# Autodesk Inventor assembly: КВ33.000.100 - Блок переключение передач
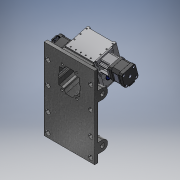
[picture p0: Inventor's stored thumbnail of the model, 180x180]
Saved by Autodesk Inventor 2019 (Build 230136000, 136)
## iProperties
Created: 2021-02-22
Part Number: КВ33.000.100 - Блок переключение передач
Material: Типовые
Document SubType Name: Assembly
Designer: Петров Иван
Author: Петров Иван
## Documents named in this file (14)
- E:\IVAN\Ivan_desktop\Kvantorium\Projects\tractor\design\КВ33.000.100 - Блок переключение передач.iam
- E:\IVAN\Ivan_desktop\Kvantorium\Projects\tractor\design\design_models\крышка КП.ipt
- E:\IVAN\Ivan_desktop\Kvantorium\Projects\tractor\design\КВ33.000.101 - Площадка крепежная.ipt
- E:\IVAN\Ivan_desktop\Kvantorium\Projects\tractor\design\КВ33.000.102 - Стенка толстая.ipt
- E:\IVAN\Ivan_desktop\Kvantorium\Projects\tractor\design\КВ33.000.103 - Стенка тонкая.ipt
- C:\Users\Петров Иван\Documents\Inventor\Content Center Files\R2019\en-US\GOST 9649-78\Washer 3 GOST 9649-78.ipt
- C:\Users\Петров Иван\Documents\Inventor\Content Center Files\R2019\en-US\Screw A2 GOST 17473-80\Screw A2.M2.5-6gx7 GOST 17473-80.ipt
- E:\IVAN\Ivan_desktop\Kvantorium\Projects\tractor\design\КВ33.000.104 - Крышка.ipt
- E:\IVAN\Ivan_desktop\Kvantorium\Projects\tractor\design\standart_components\Вал.ipt
- E:\IVAN\Ivan_desktop\Kvantorium\Projects\tractor\design\standart_components\Подшипник 626Z.ipt
- E:\IVAN\Ivan_desktop\Kvantorium\Projects\tractor\design\КВ33.000.105 - Заслонка.ipt
- E:\IVAN\Ivan_desktop\Kvantorium\Projects\tractor\design\standart_components\nema 17 motor.ipt
- E:\IVAN\Ivan_desktop\Kvantorium\Projects\tractor\design\КВ33.000.106 - Муфта.ipt
- E:\IVAN\Ivan_desktop\Kvantorium\Projects\tractor\design\КВ33.000.107 - Крепеж мотора.ipt
## Components (74 placed, 13 different names)
1. крышка КП:1 — Mate:1, Mate:8, Mate:9
2. КВ33.000.101 - Площадка крепежная:1 — Mate:1, Mate:3, Angle:1, Mate:4, Mate:6, Mate:8, Mate:9, Mate:21, Mate:27, Mate:28, Mate:37
3. КВ33.000.102 - Стенка толстая:1 — Mate:3, Angle:1, Insert:6, Insert:7, Insert:8, Insert:9, Insert:10, Mate:14, Mate:15, Mate:16, Mate:17, Mate:20, Mate:23, Mate:25, Mate:26, Mate:38, Angle:2, Mate:47
4. КВ33.000.102 - Стенка толстая:2 — Mate:4, Insert:1, Insert:2, Insert:3, Insert:4, Insert:5, Flush:4, Mate:10, Mate:11, Mate:12, Mate:13, Flush:5, Mate:28, Mate:37, Mate:42
5. КВ33.000.103 - Стенка тонкая:2 — Mate:6, Insert:22, Insert:23, Insert:24, Insert:25, Insert:26, Insert:27, Insert:28, Insert:29, Insert:30, Insert:31, Insert:32, Mate:21, Mate:38, Flush:10
6. КВ33.000.104 - Крышка:1 — Flush:4
7. Подшипник 626Z:1 — Mate:10, Mate:11, Mate:18
8. Подшипник 626Z:2 — Mate:14, Mate:15
9. Подшипник 626Z:3 — Mate:16, Mate:17
10. Подшипник 626Z:4 — Mate:12, Mate:13, Mate:19
11. Вал:1 — Mate:18, Flush:5, Flush:6, Mate:31, Mate:40, Rotation:2
12. Вал:2 — Mate:19, Flush:6, Mate:22, Mate:29, Mate:30, Rotation:1
13. КВ33.000.105 - Заслонка:1 — Mate:20
14. nema 17 motor:1 — Mate:22, Mate:23, Mate:48
15. nema 17 motor:2 — Mate:43, Mate:44, Mate:45
16. КВ33.000.103 - Стенка тонкая:3 — Mate:25, Mate:26, Mate:27, Flush:11
17. КВ33.000.106 - Муфта:1 — Mate:29, Mate:30, Mate:46, Rotation:1
18. КВ33.000.106 - Муфта:2 — Mate:31, Mate:40, Mate:41, Rotation:2
19. КВ33.000.107 - Крепеж мотора:1 — Angle:2, Flush:11, Mate:46, Mate:47, Mate:48
20. КВ33.000.107 - Крепеж мотора:2 — Mate:41, Mate:42, Flush:10, Mate:43, Mate:44, Mate:45
21. Washer GOST 9649-78 3:1 — Insert:1, Insert:49
22. Washer GOST 9649-78 3:2 — Insert:2, Insert:50
23. Washer GOST 9649-78 3:3 — Insert:3, Insert:51
24. Washer GOST 9649-78 3:4 — Insert:4, Insert:52
25. Washer GOST 9649-78 3:5 — Insert:5, Insert:53
26. Washer GOST 9649-78 3:6 — Insert:6, Insert:33
27. Washer GOST 9649-78 3:7 — Insert:7, Insert:34
28. Washer GOST 9649-78 3:8 — Insert:8, Insert:35
29. Washer GOST 9649-78 3:9 — Insert:9, Insert:36
30. Washer GOST 9649-78 3:10 — Insert:10, Insert:37
31. Washer GOST 9649-78 3:11 — Insert:42
32. Washer GOST 9649-78 3:12 — Insert:40
33. Washer GOST 9649-78 3:13 — Insert:41
34. Washer GOST 9649-78 3:14 — Insert:39
35. Washer GOST 9649-78 3:15 — Insert:38
36. Washer GOST 9649-78 3:16 — Insert:45
37. Washer GOST 9649-78 3:17 — Insert:44
38. Washer GOST 9649-78 3:18 — Insert:43
39. Washer GOST 9649-78 3:19 — Insert:46
40. Washer GOST 9649-78 3:20 — Insert:47
41. Washer GOST 9649-78 3:21 — Insert:48
42. Washer GOST 9649-78 3:22 — Insert:22
43. Washer GOST 9649-78 3:23 — Insert:23
44. Washer GOST 9649-78 3:24 — Insert:24
45. Washer GOST 9649-78 3:25 — Insert:25
46. Washer GOST 9649-78 3:26 — Insert:26
47. Washer GOST 9649-78 3:27 — Insert:27
48. Washer GOST 9649-78 3:28 — Insert:28
49. Washer GOST 9649-78 3:29 — Insert:29
50. Washer GOST 9649-78 3:30 — Insert:30, Insert:54
51. Washer GOST 9649-78 3:31 — Insert:31
52. Washer GOST 9649-78 3:32 — Insert:32
53. Screw A2 GOST 17473-80 M2.5-6gx7:1 — Insert:33
54. Screw A2 GOST 17473-80 M2.5-6gx7:2 — Insert:34
55. Screw A2 GOST 17473-80 M2.5-6gx7:3 — Insert:35
56. Screw A2 GOST 17473-80 M2.5-6gx7:4 — Insert:36
57. Screw A2 GOST 17473-80 M2.5-6gx7:5 — Insert:37
58. Screw A2 GOST 17473-80 M2.5-6gx7:6 — Insert:38
59. Screw A2 GOST 17473-80 M2.5-6gx7:7 — Insert:39
60. Screw A2 GOST 17473-80 M2.5-6gx7:8 — Insert:40
61. Screw A2 GOST 17473-80 M2.5-6gx7:9 — Insert:41
62. Screw A2 GOST 17473-80 M2.5-6gx7:10 — Insert:42
63. Screw A2 GOST 17473-80 M2.5-6gx7:11 — Insert:43
64. Screw A2 GOST 17473-80 M2.5-6gx7:12 — Insert:44
65. Screw A2 GOST 17473-80 M2.5-6gx7:13 — Insert:45
66. Screw A2 GOST 17473-80 M2.5-6gx7:14 — Insert:46
67. Screw A2 GOST 17473-80 M2.5-6gx7:15 — Insert:47
68. Screw A2 GOST 17473-80 M2.5-6gx7:16 — Insert:48
69. Screw A2 GOST 17473-80 M2.5-6gx7:17 — Insert:49
70. Screw A2 GOST 17473-80 M2.5-6gx7:18 — Insert:50
71. Screw A2 GOST 17473-80 M2.5-6gx7:19 — Insert:51
72. Screw A2 GOST 17473-80 M2.5-6gx7:20 — Insert:52
73. Screw A2 GOST 17473-80 M2.5-6gx7:21 — Insert:53
74. Screw A2 GOST 17473-80 M2.5-6gx7:22 — Insert:54
## Relationships (90: Insert 43, Mate 38, Flush 5, Angle 2, RelateRotation 2)
- Mate:1: крышка КП:1 ↔ КВ33.000.101 - Площадка крепежная:1
- Mate:3: КВ33.000.101 - Площадка крепежная:1 ↔ КВ33.000.102 - Стенка толстая:1
- Angle:1 (0 deg): КВ33.000.101 - Площадка крепежная:1 ↔ КВ33.000.102 - Стенка толстая:1
- Mate:4: КВ33.000.101 - Площадка крепежная:1 ↔ КВ33.000.102 - Стенка толстая:2
- Mate:6: КВ33.000.101 - Площадка крепежная:1 ↔ КВ33.000.103 - Стенка тонкая:2
- Insert:1: КВ33.000.102 - Стенка толстая:2 ↔ Washer GOST 9649-78 3:1
- Insert:2: КВ33.000.102 - Стенка толстая:2 ↔ Washer GOST 9649-78 3:2
- Insert:3: КВ33.000.102 - Стенка толстая:2 ↔ Washer GOST 9649-78 3:3
- Insert:4: КВ33.000.102 - Стенка толстая:2 ↔ Washer GOST 9649-78 3:4
- Insert:5: КВ33.000.102 - Стенка толстая:2 ↔ Washer GOST 9649-78 3:5
- Insert:6: КВ33.000.102 - Стенка толстая:1 ↔ Washer GOST 9649-78 3:6
- Insert:7: КВ33.000.102 - Стенка толстая:1 ↔ Washer GOST 9649-78 3:7
- Insert:8: КВ33.000.102 - Стенка толстая:1 ↔ Washer GOST 9649-78 3:8
- Insert:9: КВ33.000.102 - Стенка толстая:1 ↔ Washer GOST 9649-78 3:9
- Insert:10: КВ33.000.102 - Стенка толстая:1 ↔ Washer GOST 9649-78 3:10
- Insert:22: КВ33.000.103 - Стенка тонкая:2 ↔ Washer GOST 9649-78 3:22
- Insert:23: КВ33.000.103 - Стенка тонкая:2 ↔ Washer GOST 9649-78 3:23
- Insert:24: КВ33.000.103 - Стенка тонкая:2 ↔ Washer GOST 9649-78 3:24
- Insert:25: КВ33.000.103 - Стенка тонкая:2 ↔ Washer GOST 9649-78 3:25
- Insert:26: КВ33.000.103 - Стенка тонкая:2 ↔ Washer GOST 9649-78 3:26
- Insert:27: КВ33.000.103 - Стенка тонкая:2 ↔ Washer GOST 9649-78 3:27
- Insert:28: КВ33.000.103 - Стенка тонкая:2 ↔ Washer GOST 9649-78 3:28
- Insert:29: КВ33.000.103 - Стенка тонкая:2 ↔ Washer GOST 9649-78 3:29
- Insert:30: КВ33.000.103 - Стенка тонкая:2 ↔ Washer GOST 9649-78 3:30
- Insert:31: КВ33.000.103 - Стенка тонкая:2 ↔ Washer GOST 9649-78 3:31
- Insert:32: КВ33.000.103 - Стенка тонкая:2 ↔ Washer GOST 9649-78 3:32
- Insert:33: Washer GOST 9649-78 3:6 ↔ Screw A2 GOST 17473-80 M2.5-6gx7:1
- Insert:34: Washer GOST 9649-78 3:7 ↔ Screw A2 GOST 17473-80 M2.5-6gx7:2
- Insert:35: Washer GOST 9649-78 3:8 ↔ Screw A2 GOST 17473-80 M2.5-6gx7:3
- Insert:36: Washer GOST 9649-78 3:9 ↔ Screw A2 GOST 17473-80 M2.5-6gx7:4
- Insert:37: Washer GOST 9649-78 3:10 ↔ Screw A2 GOST 17473-80 M2.5-6gx7:5
- Insert:38: Washer GOST 9649-78 3:15 ↔ Screw A2 GOST 17473-80 M2.5-6gx7:6
- Insert:39: Washer GOST 9649-78 3:14 ↔ Screw A2 GOST 17473-80 M2.5-6gx7:7
- Insert:40: Washer GOST 9649-78 3:12 ↔ Screw A2 GOST 17473-80 M2.5-6gx7:8
- Insert:41: Washer GOST 9649-78 3:13 ↔ Screw A2 GOST 17473-80 M2.5-6gx7:9
- Insert:42: Washer GOST 9649-78 3:11 ↔ Screw A2 GOST 17473-80 M2.5-6gx7:10
- Insert:43: Washer GOST 9649-78 3:18 ↔ Screw A2 GOST 17473-80 M2.5-6gx7:11
- Insert:44: Washer GOST 9649-78 3:17 ↔ Screw A2 GOST 17473-80 M2.5-6gx7:12
- Insert:45: Washer GOST 9649-78 3:16 ↔ Screw A2 GOST 17473-80 M2.5-6gx7:13
- Insert:46: Washer GOST 9649-78 3:19 ↔ Screw A2 GOST 17473-80 M2.5-6gx7:14
- Insert:47: Washer GOST 9649-78 3:20 ↔ Screw A2 GOST 17473-80 M2.5-6gx7:15
- Insert:48: Washer GOST 9649-78 3:21 ↔ Screw A2 GOST 17473-80 M2.5-6gx7:16
- Insert:49: Washer GOST 9649-78 3:1 ↔ Screw A2 GOST 17473-80 M2.5-6gx7:17
- Insert:50: Washer GOST 9649-78 3:2 ↔ Screw A2 GOST 17473-80 M2.5-6gx7:18
- Insert:51: Washer GOST 9649-78 3:3 ↔ Screw A2 GOST 17473-80 M2.5-6gx7:19
- Insert:52: Washer GOST 9649-78 3:4 ↔ Screw A2 GOST 17473-80 M2.5-6gx7:20
- Insert:53: Washer GOST 9649-78 3:5 ↔ Screw A2 GOST 17473-80 M2.5-6gx7:21
- Insert:54: Washer GOST 9649-78 3:30 ↔ Screw A2 GOST 17473-80 M2.5-6gx7:22
- Flush:4: КВ33.000.102 - Стенка толстая:2 ↔ КВ33.000.104 - Крышка:1
- Mate:8: крышка КП:1 ↔ КВ33.000.101 - Площадка крепежная:1
- Mate:9: крышка КП:1 ↔ КВ33.000.101 - Площадка крепежная:1
- Mate:10: КВ33.000.102 - Стенка толстая:2 ↔ Подшипник 626Z:1
- Mate:11: КВ33.000.102 - Стенка толстая:2 ↔ Подшипник 626Z:1
- Mate:12: КВ33.000.102 - Стенка толстая:2 ↔ Подшипник 626Z:4
- Mate:13: КВ33.000.102 - Стенка толстая:2 ↔ Подшипник 626Z:4
- Mate:14: КВ33.000.102 - Стенка толстая:1 ↔ Подшипник 626Z:2
- Mate:15: КВ33.000.102 - Стенка толстая:1 ↔ Подшипник 626Z:2
- Mate:16: КВ33.000.102 - Стенка толстая:1 ↔ Подшипник 626Z:3
- Mate:17: КВ33.000.102 - Стенка толстая:1 ↔ Подшипник 626Z:3
- Mate:18: Подшипник 626Z:1 ↔ Вал:1
- Flush:5 (-7.5 mm): КВ33.000.102 - Стенка толстая:2 ↔ Вал:1
- Mate:19: Подшипник 626Z:4 ↔ Вал:2
- Flush:6: Вал:1 ↔ Вал:2
- Mate:20: КВ33.000.102 - Стенка толстая:1 ↔ КВ33.000.105 - Заслонка:1
- Mate:21: КВ33.000.101 - Площадка крепежная:1 ↔ КВ33.000.103 - Стенка тонкая:2
- Mate:22: Вал:2 ↔ nema 17 motor:1
- Mate:23 (32 mm): КВ33.000.102 - Стенка толстая:1 ↔ nema 17 motor:1
- Mate:25: КВ33.000.102 - Стенка толстая:1 ↔ КВ33.000.103 - Стенка тонкая:3
- Mate:26: КВ33.000.102 - Стенка толстая:1 ↔ КВ33.000.103 - Стенка тонкая:3
- Mate:27: КВ33.000.101 - Площадка крепежная:1 ↔ КВ33.000.103 - Стенка тонкая:3
- Mate:28: КВ33.000.101 - Площадка крепежная:1 ↔ КВ33.000.102 - Стенка толстая:2
- Mate:29: Вал:2 ↔ КВ33.000.106 - Муфта:1
- Mate:30: Вал:2 ↔ КВ33.000.106 - Муфта:1
- Mate:31: Вал:1 ↔ КВ33.000.106 - Муфта:2
- Mate:37: КВ33.000.101 - Площадка крепежная:1 ↔ КВ33.000.102 - Стенка толстая:2
- Mate:38: КВ33.000.102 - Стенка толстая:1 ↔ КВ33.000.103 - Стенка тонкая:2
- Mate:40: Вал:1 ↔ КВ33.000.106 - Муфта:2
- Mate:41: КВ33.000.106 - Муфта:2 ↔ КВ33.000.107 - Крепеж мотора:2
- Mate:42: КВ33.000.102 - Стенка толстая:2 ↔ КВ33.000.107 - Крепеж мотора:2
- Flush:10: КВ33.000.103 - Стенка тонкая:2 ↔ КВ33.000.107 - Крепеж мотора:2
- Mate:43: nema 17 motor:2 ↔ КВ33.000.107 - Крепеж мотора:2
- Mate:44: nema 17 motor:2 ↔ КВ33.000.107 - Крепеж мотора:2
- Mate:45: nema 17 motor:2 ↔ КВ33.000.107 - Крепеж мотора:2
- Angle:2 (0 deg): КВ33.000.102 - Стенка толстая:1 ↔ КВ33.000.107 - Крепеж мотора:1
- Flush:11: КВ33.000.103 - Стенка тонкая:3 ↔ КВ33.000.107 - Крепеж мотора:1
- Mate:46: КВ33.000.106 - Муфта:1 ↔ КВ33.000.107 - Крепеж мотора:1
- Mate:47: КВ33.000.102 - Стенка толстая:1 ↔ КВ33.000.107 - Крепеж мотора:1
- Mate:48: nema 17 motor:1 ↔ КВ33.000.107 - Крепеж мотора:1
- Rotation:1 [RelateRotation] (1 ul): Вал:2 ↔ КВ33.000.106 - Муфта:1
- Rotation:2 [RelateRotation] (1 ul): Вал:1 ↔ КВ33.000.106 - Муфта:2
